# Autodesk Inventor assembly: S8x6
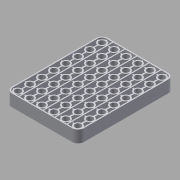
[picture p0: Inventor's stored thumbnail of the model, 180x180]
Saved by Autodesk Inventor 2019.3 (Build 233278000, 278)
## iProperties
Created: 2019-01-31
Part Number: S8x6
Document SubType Name: Assembly
Designer: Varga Daniel
Author: Varga Daniel
## Documents named in this file (10)
- C:\!_Dani\!_cloud\OneDrive\!_munka\Revolution\RevvyDemoKit\Structural parts\Beams\Straight Beams\S3+x3+.iam
- C:\!_Dani\!_cloud\OneDrive\!_munka\Revolution\RevvyDemoKit\Structural parts\Beams\beam_side_part.ipt
- C:\!_Dani\!_cloud\OneDrive\!_munka\Revolution\RevvyDemoKit\Structural parts\Beams\beam_inner_part.ipt
- C:\!_Dani\!_cloud\OneDrive\!_munka\Revolution\RevvyDemoKit\Structural parts\Beams\beam_corner_part.ipt
- C:\!_Dani\!_cloud\OneDrive\!_munka\Revolution\RevvyDemoKit\Structural parts\Beams\beam_top_bot_part.ipt
- S3x4.iam
- S4x3.iam
- S4x4.iam
- S8x4.iam
- S8x6.iam
## Components (48 placed, 4 different names)
1. beam_corner_part:1 — Flush:1, Flush:2, Mate:1, Flush:3, Flush:4, Mate:2, Flush:5, Flush:6, Flush:11, Flush:12, Mate:5, Mate:8
2. beam_corner_part:2 — Mate:1, Flush:3, Flush:4
3. beam_corner_part:3 — Flush:11, Flush:12, Mate:5, Flush:13, Flush:14, Mate:6, Flush:15, Flush:16, Mate:7
4. beam_corner_part:4 — Flush:13, Flush:14, Mate:6
5. beam_top_bot_part:1 — Flush:1, Flush:2, Mate:2
6. beam_top_bot_part:4
7. beam_top_bot_part:5
8. beam_top_bot_part:6
9. beam_top_bot_part:3 — Flush:15, Flush:16, Mate:7
10. beam_top_bot_part:9
11. beam_top_bot_part:10
12. beam_top_bot_part:11
13. beam_side_part:2 — Flush:7, Flush:8, Mate:3
14. beam_side_part:1 — Flush:5, Flush:6, Flush:7, Flush:8, Mate:3, Flush:9, Flush:10, Mate:4, Mate:8
15. beam_side_part:3
16. beam_side_part:4
17. beam_side_part:5
18. beam_side_part:6
19. beam_side_part:7
20. beam_side_part:8
21. beam_side_part:9
22. beam_side_part:10
23. beam_side_part:11
24. beam_side_part:12
25. beam_inner_part:1 — Flush:9, Flush:10, Mate:4
26. beam_inner_part:6
27. beam_inner_part:7
28. beam_inner_part:8
29. beam_inner_part:5
30. beam_inner_part:11
31. beam_inner_part:12
32. beam_inner_part:13
33. beam_inner_part:16
34. beam_inner_part:17
35. beam_inner_part:18
36. beam_inner_part:19
37. beam_inner_part:22
38. beam_inner_part:23
39. beam_inner_part:24
40. beam_inner_part:25
41. beam_inner_part:28
42. beam_inner_part:29
43. beam_inner_part:30
44. beam_inner_part:31
45. beam_inner_part:32
46. beam_inner_part:33
47. beam_inner_part:34
48. beam_inner_part:35
## Component patterns: (4 elements, first: beam_top_bot_part:1), (4 elements, first: beam_top_bot_part:3), (6 elements, first: beam_side_part:2 + beam_side_part:1), (4 elements, first: beam_inner_part:1), Component Pattern 6:2 (4 elements), Component Pattern 6:3 (4 elements), Component Pattern 6:4 (4 elements), Component Pattern 6:5 (4 elements), Component Pattern 6:6 (4 elements)
## Relationships (24: Flush 16, Mate 8)
- Flush:1: beam_corner_part:1 ↔ beam_top_bot_part:1
- Flush:2: beam_corner_part:1 ↔ beam_top_bot_part:1
- Mate:1 (40 mm): beam_corner_part:1 ↔ beam_corner_part:2
- Flush:3: beam_corner_part:1 ↔ beam_corner_part:2
- Flush:4: beam_corner_part:1 ↔ beam_corner_part:2
- Mate:2: beam_corner_part:1 ↔ beam_top_bot_part:1
- Flush:5: beam_corner_part:1 ↔ beam_side_part:1
- Flush:6: beam_corner_part:1 ↔ beam_side_part:1
- Flush:7: beam_side_part:2 ↔ beam_side_part:1
- Flush:8: beam_side_part:2 ↔ beam_side_part:1
- Mate:3 (40 mm): beam_side_part:2 ↔ beam_side_part:1
- Flush:9: beam_side_part:1 ↔ beam_inner_part:1
- Flush:10: beam_side_part:1 ↔ beam_inner_part:1
- Mate:4: beam_side_part:1 ↔ beam_inner_part:1
- Flush:11: beam_corner_part:1 ↔ beam_corner_part:3
- Flush:12: beam_corner_part:1 ↔ beam_corner_part:3
- Mate:5 (60 mm): beam_corner_part:1 ↔ beam_corner_part:3
- Flush:13: beam_corner_part:3 ↔ beam_corner_part:4
- Flush:14: beam_corner_part:3 ↔ beam_corner_part:4
- Mate:6 (40 mm): beam_corner_part:3 ↔ beam_corner_part:4
- Flush:15: beam_corner_part:3 ↔ beam_top_bot_part:3
- Flush:16: beam_corner_part:3 ↔ beam_top_bot_part:3
- Mate:7: beam_corner_part:3 ↔ beam_top_bot_part:3
- Mate:8: beam_corner_part:1 ↔ beam_side_part:1
